# Autodesk Inventor assembly: 円盤
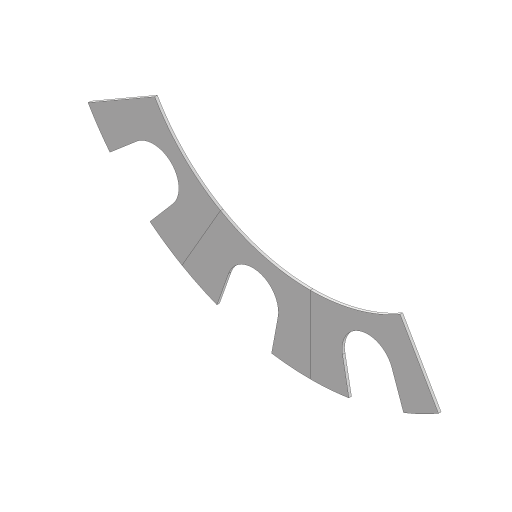
[picture p0: Inventor's stored thumbnail of the model, 512x512]
Saved by Autodesk Inventor 2023 (Build 270158000, 158)
## iProperties
Created: 2022-09-02
Part Number: 円盤
Document SubType Name: Assembly
Designer: monst
Author: monst
## Documents named in this file (2)
- D:\VENUSFOUNTAIN\Assets\円盤.iam
- D:\VENUSFOUNTAIN\Assets\円盤1.ipt
## Components (3 placed, 1 different names)
1. 円盤1:1 — メイト:1, メイト:2, フラッシュ:1, フラッシュ:2, メイト:3, メイト:4
2. 円盤1:2 — フラッシュ:2, メイト:3, メイト:4
3. 円盤1:3 — メイト:1, メイト:2, フラッシュ:1
## Relationships (6: Mate 4, Flush 2)
- メイト:1 [Mate]: 円盤1:1 ↔ 円盤1:3
- メイト:2 [Mate]: 円盤1:1 ↔ 円盤1:3
- フラッシュ:1 [Flush]: 円盤1:1 ↔ 円盤1:3
- フラッシュ:2 [Flush]: 円盤1:1 ↔ 円盤1:2
- メイト:3 [Mate]: 円盤1:1 ↔ 円盤1:2
- メイト:4 [Mate]: 円盤1:1 ↔ 円盤1:2
